# Autodesk Inventor assembly: StepperSystem
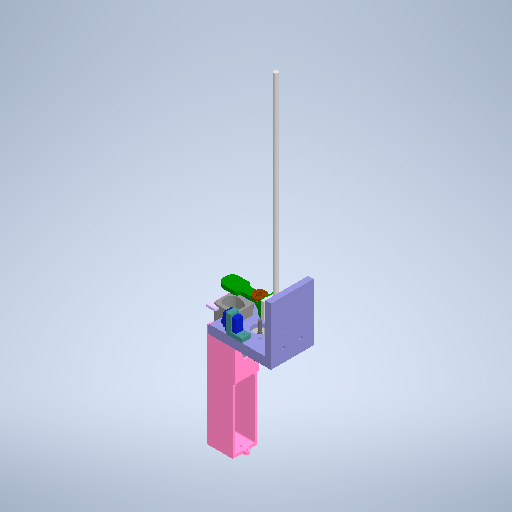
[picture p0: Inventor's stored thumbnail of the model, 512x512]
Saved by Autodesk Inventor 2025.1 (Build 291241000, 241)
## iProperties
Created: 2025-01-26
Part Number: StepperSystem
Document SubType Name: Assembly
Designer: 13156
Author: 13156
## Documents named in this file (13)
- C:\Users\13156\OneDrive - Binghamton University\Documents\GitHub\Perovskite-Automated-Synthesis-System\CAD\Pipette\StepperSystem.iam
- C:\Users\13156\OneDrive - Binghamton University\Documents\GitHub\Perovskite-Automated-Synthesis-System\CAD\Pipette\HolderWStepper.ipt
- C:\Users\13156\OneDrive - Binghamton University\Documents\GitHub\Perovskite-Automated-Synthesis-System\CAD\Non 3D Printed Parts\Linear Rails\8mm Linear Rod.ipt
- C:\Users\13156\OneDrive - Binghamton University\Documents\GitHub\Perovskite-Automated-Synthesis-System\CAD\Non 3D Printed Parts\Linear Rails\Linear Bearing 8mm Square.ipt
- C:\Users\13156\OneDrive - Binghamton University\Documents\GitHub\Perovskite-Automated-Synthesis-System\CAD\Pipette\Actuator.ipt
- C:\Users\13156\OneDrive - Binghamton University\Documents\GitHub\Perovskite-Automated-Synthesis-System\CAD\Pipette\PipetteStand.ipt
- C:\Users\13156\OneDrive - Binghamton University\Documents\GitHub\Perovskite-Automated-Synthesis-System\CAD\Non 3D Printed Parts\Motors and Servos\SG90 Servo.ipt
- C:\Users\13156\OneDrive - Binghamton University\Documents\GitHub\Perovskite-Automated-Synthesis-System\CAD\Pipette\GrabberArm.ipt
- C:\Users\13156\OneDrive - Binghamton University\Documents\GitHub\Perovskite-Automated-Synthesis-System\CAD\Pipette\SLEEVE.ipt
- C:\Users\13156\OneDrive - Binghamton University\Documents\GitHub\Perovskite-Automated-Synthesis-System\CAD\Non 3D Printed Parts\Leadscrew.ipt
- C:\Users\13156\OneDrive - Binghamton University\Documents\GitHub\Perovskite-Automated-Synthesis-System\CAD\Non 3D Printed Parts\Linear Rails\Linear Rod Holder SK8.ipt
- C:\Users\13156\OneDrive - Binghamton University\Documents\GitHub\Perovskite-Automated-Synthesis-System\CAD\Non 3D Printed Parts\Motors and Servos\NEMA17 Stepper Motor - 26 mm.ipt
- C:\Users\13156\OneDrive - Binghamton University\Documents\GitHub\Perovskite-Automated-Synthesis-System\CAD\Pipette\ServoHolder.ipt
## Components (13 placed, 12 different names)
1. HolderWStepper:1 — Mate:9, Mate:13, Mate:14, Mate:15, Mate:16, Mate:25, Mate:26, Mate:38, Mate:39, Mate:40, Flush:4, Mate:46, Mate:47, Mate:50, Mate:51, Mate:54
2. 8mm Linear Rod:1 — Mate:21, Flush:4, Mate:48
3. Linear Bearing 8mm Square:1 — Mate:21, Mate:28, Mate:29, Mate:30, Mate:49
4. Actuator:1 — Mate:28, Mate:29, Mate:30, Mate:31, Mate:32, Mate:33, Mate:49
5. PipetteStand:1 — Mate:1, Mate:2, Mate:3, Mate:4, Mate:6
6. SG90 Servo:1 — Mate:38, Mate:39, Mate:40, Mate:44
7. GrabberArm:1 — Mate:44
8. Leadscrew:1 — Mate:31, Mate:32, Mate:33
9. Linear Rod Holder SK8:1 — Mate:13, Mate:14, Mate:15, Mate:16, Mate:48
10. SG90 Servo:3 — Mate:52, Mate:55
11. NEMA17 Stepper Motor - 26 mm:2 — Mate:9, Mate:25, Mate:26
12. SLEEVE:1 — Mate:4, Mate:6, Mate:46, Mate:47, Mate:54
13. ServoHolder:1 — Mate:50, Mate:51, Mate:52, Mate:55
## Relationships (33: Mate 32, Flush 1)
- Mate:1: PipetteStand:1
- Mate:2: PipetteStand:1
- Mate:3: PipetteStand:1
- Mate:4: PipetteStand:1 ↔ SLEEVE:1
- Mate:6 (0.5 mm): PipetteStand:1 ↔ SLEEVE:1
- Mate:9: HolderWStepper:1 ↔ NEMA17 Stepper Motor - 26 mm:2
- Mate:13: HolderWStepper:1 ↔ Linear Rod Holder SK8:1
- Mate:14: HolderWStepper:1 ↔ Linear Rod Holder SK8:1
- Mate:15: HolderWStepper:1 ↔ Linear Rod Holder SK8:1
- Mate:16: HolderWStepper:1 ↔ Linear Rod Holder SK8:1
- Mate:21: 8mm Linear Rod:1 ↔ Linear Bearing 8mm Square:1
- Mate:25: HolderWStepper:1 ↔ NEMA17 Stepper Motor - 26 mm:2
- Mate:26: HolderWStepper:1 ↔ NEMA17 Stepper Motor - 26 mm:2
- Mate:28: Linear Bearing 8mm Square:1 ↔ Actuator:1
- Mate:29: Linear Bearing 8mm Square:1 ↔ Actuator:1
- Mate:30: Linear Bearing 8mm Square:1 ↔ Actuator:1
- Mate:31: Actuator:1 ↔ Leadscrew:1
- Mate:32: Actuator:1 ↔ Leadscrew:1
- Mate:33: Actuator:1 ↔ Leadscrew:1
- Mate:38: HolderWStepper:1 ↔ SG90 Servo:1
- Mate:39: HolderWStepper:1 ↔ SG90 Servo:1
- Mate:40: HolderWStepper:1 ↔ SG90 Servo:1
- Mate:44: SG90 Servo:1 ↔ GrabberArm:1
- Flush:4: HolderWStepper:1 ↔ 8mm Linear Rod:1
- Mate:46: HolderWStepper:1 ↔ SLEEVE:1
- Mate:47: HolderWStepper:1 ↔ SLEEVE:1
- Mate:48: 8mm Linear Rod:1 ↔ Linear Rod Holder SK8:1
- Mate:49: Linear Bearing 8mm Square:1 ↔ Actuator:1
- Mate:50: HolderWStepper:1 ↔ ServoHolder:1
- Mate:51: HolderWStepper:1 ↔ ServoHolder:1
- Mate:52: SG90 Servo:3 ↔ ServoHolder:1
- Mate:54: HolderWStepper:1 ↔ SLEEVE:1
- Mate:55: SG90 Servo:3 ↔ ServoHolder:1
